# Autodesk Inventor assembly: plane
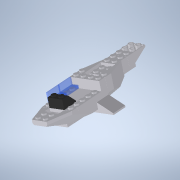
[picture p0: Inventor's stored thumbnail of the model, 180x180]
Saved by Autodesk Inventor 2021 (Build 250183000, 183)
## iProperties
Created: 2021-02-18
Part Number: plane
Document SubType Name: Assembly
Designer: bagal
Author: bagal
## Documents named in this file (18)
- C:\Users\bagal\Desktop\inventor models\airplane\plane.iam
- C:\Users\bagal\Desktop\inventor models\airplane\3975.ipt
- C:\Users\bagal\Desktop\inventor models\airplane\3710.ipt
- C:\Users\bagal\Desktop\inventor models\airplane\3022.ipt
- C:\Users\bagal\Desktop\inventor models\airplane\3024.ipt
- C:\Users\bagal\Desktop\inventor models\airplane\3298.ipt
- C:\Users\bagal\Desktop\inventor models\airplane\3623.ipt
- C:\Users\bagal\Desktop\inventor models\airplane\3023.ipt
- C:\Users\bagal\Desktop\inventor models\airplane\4856.ipt
- C:\Users\bagal\Desktop\inventor models\airplane\3666.ipt
- C:\Users\bagal\Desktop\inventor models\airplane\4855.ipt
- C:\Users\bagal\Desktop\inventor models\airplane\4859.ipt
- C:\Users\bagal\Desktop\inventor models\airplane\3003.ipt
- C:\Users\bagal\Desktop\inventor models\airplane\3747.ipt
- C:\Users\bagal\Desktop\inventor models\airplane\2399.ipt
- C:\Users\bagal\Desktop\inventor models\airplane\3010.ipt
- C:\Users\bagal\Desktop\inventor models\airplane\3039pc4.ipt
- C:\Users\bagal\Desktop\inventor models\airplane\4865.ipt
## Components (25 placed, 17 different names)
1. 3975:1 — Mate:1, Mate:2, Flush:1, Mate:4, Flush:6, Flush:7, Flush:9, Mate:15, Flush:10
2. 3710:1 — Mate:1, Mate:2, Mate:3, Flush:2, Flush:3, Mate:5, Flush:4, Mate:6, Flush:5
3. 3022:1 — Flush:1, Mate:3, Mate:4, Mate:8, Mate:9
4. 3024:1 — Flush:4, Mate:6, Flush:5, Mate:10
5. 3024:2 — Flush:2, Flush:3, Mate:5, Mate:7, Mate:16, Flush:11, Flush:13
6. 3298:1 — Mate:7, Mate:8, Flush:7, Mate:11, Mate:12, Mate:22
7. 3298:2 — Mate:9, Flush:6, Mate:10, Mate:13, Mate:14, Flush:14
8. 3623:1 — Mate:11, Mate:12, Flush:12, Flush:13, Mate:17, Flush:15
9. 3623:2 — Mate:13, Mate:14, Flush:14, Mate:19
10. 3023:1 — Flush:9, Mate:15, Flush:10
11. 4856:1 — Mate:16, Flush:11, Flush:12, Mate:18, Mate:20, Flush:16, Mate:23, Mate:25, Mate:27, Mate:28
12. 3666:1 — Mate:19, Mate:20, Flush:16, Flush:17, Mate:30, Mate:42, Mate:46, Mate:48
13. 3666:2 — Mate:17, Flush:15, Mate:18, Mate:21, Mate:24, Flush:18, Mate:39
14. 4855:1 — Mate:21, Mate:22, Flush:17, Mate:29, Mate:31, Flush:23
15. 4859:1 — Mate:23, Mate:26, Mate:27, Mate:28
16. 4859:2 — Mate:29, Mate:30, Mate:31, Flush:19, Mate:32, Flush:20, Mate:33, Mate:34, Mate:37
17. 3710:2 — Mate:24, Mate:25, Flush:18, Mate:26, Flush:25, Mate:41
18. 3022:2 — Flush:19, Mate:32, Flush:20, Flush:21, Mate:35
19. 3003:1 — Mate:33, Mate:34, Flush:21, Flush:22, Mate:36, Mate:38
20. 3747:1 — Mate:35, Flush:22, Mate:36
21. 2399:1 — Mate:37, Flush:23, Mate:38, Mate:40, Flush:24
22. 3010:1 — Mate:39, Mate:40, Flush:24, Mate:47, Flush:26
23. 3039pc4:1 — Flush:25, Mate:41, Mate:42
24. 4865:1 — Mate:46, Flush:27, Mate:49
25. 4865:2 — Mate:47, Mate:48, Flush:26, Flush:27, Mate:49
## Relationships (72: Mate 46, Flush 26)
- Mate:1: 3975:1 ↔ 3710:1
- Mate:2: 3975:1 ↔ 3710:1
- Flush:1: 3975:1 ↔ 3022:1
- Mate:3: 3710:1 ↔ 3022:1
- Mate:4: 3975:1 ↔ 3022:1
- Flush:2: 3710:1 ↔ 3024:2
- Flush:3: 3710:1 ↔ 3024:2
- Mate:5: 3710:1 ↔ 3024:2
- Flush:4: 3710:1 ↔ 3024:1
- Mate:6: 3710:1 ↔ 3024:1
- Flush:5: 3710:1 ↔ 3024:1
- Mate:7: 3024:2 ↔ 3298:1
- Mate:8: 3022:1 ↔ 3298:1
- Mate:9: 3022:1 ↔ 3298:2
- Flush:6: 3975:1 ↔ 3298:2
- Mate:10: 3024:1 ↔ 3298:2
- Flush:7: 3975:1 ↔ 3298:1
- Mate:11: 3298:1 ↔ 3623:1
- Mate:12: 3298:1 ↔ 3623:1
- Mate:13: 3298:2 ↔ 3623:2
- Mate:14: 3298:2 ↔ 3623:2
- Flush:9: 3975:1 ↔ 3023:1
- Mate:15: 3975:1 ↔ 3023:1
- Flush:10: 3975:1 ↔ 3023:1
- Mate:16: 3024:2 ↔ 4856:1
- Flush:11: 3024:2 ↔ 4856:1
- Flush:12: 3623:1 ↔ 4856:1
- Flush:13: 3024:2 ↔ 3623:1
- Flush:14: 3298:2 ↔ 3623:2
- Mate:17: 3623:1 ↔ 3666:2
- Flush:15: 3623:1 ↔ 3666:2
- Mate:18: 4856:1 ↔ 3666:2
- Mate:19: 3623:2 ↔ 3666:1
- Mate:20: 4856:1 ↔ 3666:1
- Flush:16: 4856:1 ↔ 3666:1
- Mate:21: 3666:2 ↔ 4855:1
- Mate:22: 3298:1 ↔ 4855:1
- Flush:17: 3666:1 ↔ 4855:1
- Mate:23: 4856:1 ↔ 4859:1
- Mate:24: 3666:2 ↔ 3710:2
- Mate:25: 4856:1 ↔ 3710:2
- Flush:18: 3666:2 ↔ 3710:2
- Mate:26: 4859:1 ↔ 3710:2
- Mate:27: 4856:1 ↔ 4859:1
- Mate:28: 4856:1 ↔ 4859:1
- Mate:29: 4855:1 ↔ 4859:2
- Mate:30: 3666:1 ↔ 4859:2
- Mate:31: 4855:1 ↔ 4859:2
- Flush:19: 4859:2 ↔ 3022:2
- Mate:32: 4859:2 ↔ 3022:2
- Flush:20: 4859:2 ↔ 3022:2
- Mate:33: 4859:2 ↔ 3003:1
- Mate:34: 4859:2 ↔ 3003:1
- Flush:21: 3022:2 ↔ 3003:1
- Mate:35: 3022:2 ↔ 3747:1
- Flush:22: 3003:1 ↔ 3747:1
- Mate:36: 3003:1 ↔ 3747:1
- Mate:37: 4859:2 ↔ 2399:1
- Flush:23: 4855:1 ↔ 2399:1
- Mate:38: 3003:1 ↔ 2399:1
- Mate:39: 3666:2 ↔ 3010:1
- Mate:40: 2399:1 ↔ 3010:1
- Flush:24: 2399:1 ↔ 3010:1
- Flush:25: 3710:2 ↔ 3039pc4:1
- Mate:41: 3710:2 ↔ 3039pc4:1
- Mate:42: 3666:1 ↔ 3039pc4:1
- Mate:46: 3666:1 ↔ 4865:1
- Mate:47: 3010:1 ↔ 4865:2
- Mate:48: 3666:1 ↔ 4865:2
- Flush:26: 3010:1 ↔ 4865:2
- Flush:27: 4865:1 ↔ 4865:2
- Mate:49: 4865:1 ↔ 4865:2
